# Autodesk Inventor assembly: Shed_Area
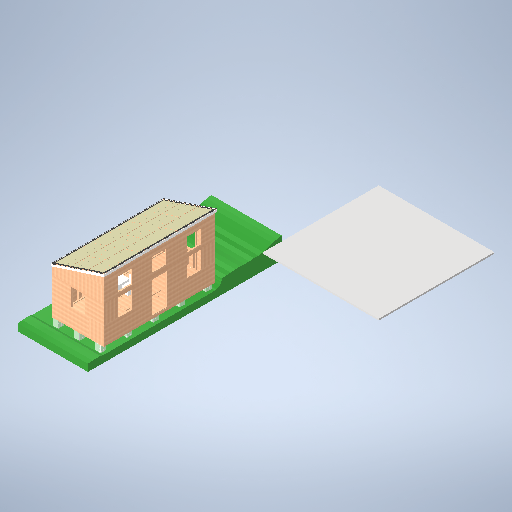
[picture p0: Inventor's stored thumbnail of the model, 512x512]
Saved by Autodesk Inventor 2025 (Build 290162010, 162A)
## iProperties
Created: 2024-08-02
Part Number: Shed_Area
Document SubType Name: Assembly
Designer: Tom
Author: Tom
## Documents named in this file (5)
- C:\Users\Tom\Documents\Inventor\Mobility\Additional_Building\Area_With_Additional_Building.iam
- C:\Users\Tom\Documents\Inventor\Mobility\Additional_Building\Slab_And_Cross_Section_Of_Foundation_Walls_Of_House.ipt
- C:\Users\Tom\Documents\Inventor\Mobility\Additional_Building\Earth.ipt
- C:\Users\Tom\Documents\Inventor\Mobility\Additional_Building\Maple_Tree.ipt
- C:\Users\Tom\Documents\Inventor\Mobility\Additional_Building\Additional_Building.iam
## Components (4 placed, 4 different names)
1. Slab_And_Cross_Section_Of_Foundation_Walls_Of_House:1 — Mate:1, Mate:2, Mate:3, Flush:3, Mate:14, Flush:6
2. Earth:1 — Mate:1, Mate:2, Mate:3, Mate:13, Flush:5
3. Maple_Tree:1 — Flush:3, Mate:13
4. Additional_Building:1 [sub-assembly] — Flush:5, Mate:14, Flush:6
## Relationships (8: Mate 5, Flush 3)
- Mate:1 (-1219.2 mm): Slab_And_Cross_Section_Of_Foundation_Walls_Of_House:1 ↔ Earth:1
- Mate:2: Slab_And_Cross_Section_Of_Foundation_Walls_Of_House:1 ↔ Earth:1
- Mate:3: Slab_And_Cross_Section_Of_Foundation_Walls_Of_House:1 ↔ Earth:1
- Flush:3 (-1117.6 mm): Slab_And_Cross_Section_Of_Foundation_Walls_Of_House:1 ↔ Maple_Tree:1
- Mate:13 (-635 mm): Earth:1 ↔ Maple_Tree:1
- Flush:5 (203.2 mm): Earth:1 ↔ Additional_Building:1
- Mate:14 (3189.2875 mm): Slab_And_Cross_Section_Of_Foundation_Walls_Of_House:1 ↔ Additional_Building:1
- Flush:6: Slab_And_Cross_Section_Of_Foundation_Walls_Of_House:1 ↔ Additional_Building:1
